# Autodesk Inventor assembly: BARR608ZZ
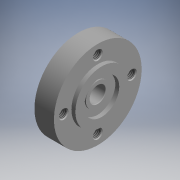
[picture p0: Inventor's stored thumbnail of the model, 180x180]
Saved by Autodesk Inventor 2017.3 (Build 213256000, 256)
## iProperties
Category: PARTsolutions
Company: MISUMI
Part Number: BARR608ZZ
Catalog Web Link: www.cadenas.de
Description: BGRRB, BGRR, BARR, SBARR, SBGRR-Bearings with Housings Pilot, Retained - Round Type
Vendor: MISUMI
Document SubType Name: Assembly
Designer: partserver
Manufacturer: MISUMI
Mass: 13.705 g
Surface Area: 75.8214 cm^2
Volume: 13.705 cm^3
Density: 1 g/cm^3
Title: BARR608ZZ
Author: Cadenas PARTsolutions
Comments: Bearings with Housings Pilot, Retained - Round Type
PSOL_IDENT_0: {$CADENAS_DATA\23d-libs\misumi\metric\12_bearing_holders\bgrrb_asmtab.prj},221 {VTYP=3D},{STYP=ASSTA
PSOL_IDENT_1: B},{NB=BARR608ZZ},{LINA=BARR608ZZ},{NN=BGRRB, BGRR, BARR, SBARR, SBGRR},{DATE=09.09.2019 15:26:55},{
PSOL_IDENT_2: GEOMDATE=18.08.2015 01:55:34},{VERSION=},{LINEID=80},{WBVAR=MATB,MATH,STH,SEALT,ALT1},{WBNUMERIC=}
PSOL_IDENT_3: {NB=BARR608ZZ},{LINA=BARR608ZZ},{KT=DUMMY},{PN=BARR608ZZ},{TYPE=BARR},{MATB=},{MATBALG=  '', 'Steel'
PSOL_IDENT_4: , 'S', 'Stainless Steel'  },{MATH=A2000},{MATH1=  'S45CE','1045 Carbon Steel Equivalent','A2000','20
PSOL_IDENT_5: 00 Aluminum Alloy'    },{STH=CA},{ST1=  'CA','Clear Anodize'  },{AC=304 Stainless Steel},{BN=608},{B
PSOL_IDENT_6: N2=608.000},{MS=0},{MS2=0.000},{SEALT=ZZ},{DD=8},{D=22},{D3=23.500},{TR=1.15},{B=7},{H=45},{T=12},{T
PSOL_IDENT_7: 1=10},{S=2},{LL1=2},{DDHH=18},{D1=27},{PCD=35},{F=0},{M=M 5 (4.3)},{DD1=8.0},{H1=4.4},{D2MIN=4.300},
PSOL_IDENT_8: {D2MAX=5.000},{NR=},{PPATH=bgrrb/bgrrb_temp.prj},{ALT1=},{SEALTALG= 'ZZ','ZZ(Double Shielded)','VV','
PSOL_IDENT_9: VV(Non-Contact Sealed Rubber Seal)','DD','DD(Contact Sealed Rubber Seal)' },{BNHALG=1},{ALT1ALG= '',
PSOL_IDENT_10: 'Bearing and Retaining Ring Assembled', '-NA'  , 'with NA (Bearing and Retaining Ring not Assembled
PSOL_IDENT_11: )'}
NB: BARR608ZZ
NN: BGRRB, BGRR, BARR, SBARR, SBGRR
NT: Bearings with Housings Pilot, Retained - Round Type
NBSYN: $PN.
LINA: BARR608ZZ
CATALOG: Misumi
PN: BARR608ZZ
MATB: Steel
MATH: 2000 Aluminum Alloy
STH: Clear Anodize
AC: 304 Stainless Steel
BN: 608
SEALT: ZZ(Double Shielded)
DD: 8
D: 22
B: 7
H: 45
T: 12
T1: 10
S: 2
LL1: 2
DDHH: 18
D1: 27
PCD: 35
F: 0
M: M 5 (4.3)
DD1: 8
H1: 4.4
ALT1: Bearing and Retaining Ring Assembled
SUPPLIER: MISUMI
ARTICLENO: BARR608ZZ
BOMINFO: BARR608ZZ
CREATOR: CADENAS GmbH
## Documents named in this file (4)
- e:\temp\worker_18\temp\exporttempdir_9308_160_tDurL\format_0\BARR608ZZ.iam
- e:\temp\worker_18\temp\exporttempdir_9308_160_tDurL\format_0\BARR608ZZ_b.ipt
- e:\temp\worker_18\temp\exporttempdir_9308_160_tDurL\format_0\bearing_608.ipt
- e:\temp\worker_18\temp\exporttempdir_9308_160_tDurL\format_0\RRING-C-INT-22.ipt
## Components (3 placed, 3 different names)
1. BARR608ZZ_b:1 — to_bearings_1_XY@1 <-> to_housing_XY@2, to_bearings_1_Z@1 <-> to_housing_Z@2, to_bearings_1_YZ@1 <-> to_housing_YZ@2, bgrrb_to_rring_XY@1 <-> rr_XY@3, bgrrb_to_rring_Z@1 <-> rr_Z@3, bgrrb_to_rring_YZ@1 <-> rr_YZ@3
2. bearing_608:1 — to_bearings_1_XY@1 <-> to_housing_XY@2, to_bearings_1_Z@1 <-> to_housing_Z@2, to_bearings_1_YZ@1 <-> to_housing_YZ@2
3. RRING-C-INT-22:1 — bgrrb_to_rring_XY@1 <-> rr_XY@3, bgrrb_to_rring_Z@1 <-> rr_Z@3, bgrrb_to_rring_YZ@1 <-> rr_YZ@3
## Relationships (6: Mate 3, Angle 2, Flush 1)
- to_bearings_1_XY@1 <-> to_housing_XY@2 [Mate] (7 mm): BARR608ZZ_b:1 ↔ bearing_608:1
- to_bearings_1_Z@1 <-> to_housing_Z@2 [Mate]: BARR608ZZ_b:1 ↔ bearing_608:1
- to_bearings_1_YZ@1 <-> to_housing_YZ@2 [Angle] (0 deg): BARR608ZZ_b:1 ↔ bearing_608:1
- bgrrb_to_rring_XY@1 <-> rr_XY@3 [Flush]: BARR608ZZ_b:1 ↔ RRING-C-INT-22:1
- bgrrb_to_rring_Z@1 <-> rr_Z@3 [Mate]: BARR608ZZ_b:1 ↔ RRING-C-INT-22:1
- bgrrb_to_rring_YZ@1 <-> rr_YZ@3 [Angle] (0 deg): BARR608ZZ_b:1 ↔ RRING-C-INT-22:1
